# Autodesk Inventor assembly: Lens_mounted
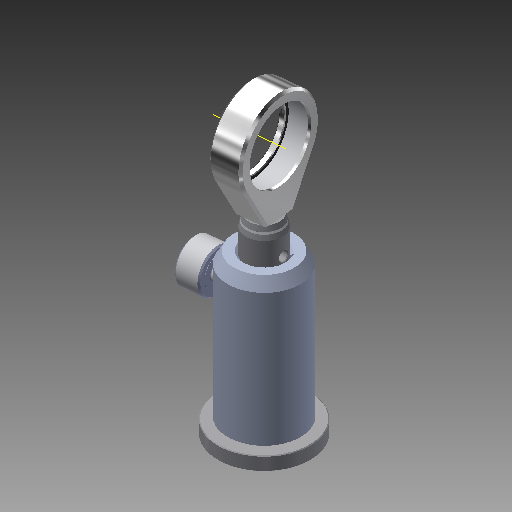
[picture p0: Inventor's stored thumbnail of the model, 512x512]
Saved by Autodesk Inventor 2017 SP1 (Build 210196100, 196)
## iProperties
Created: 2016-01-14
Part Number: Lens_mounted
Document SubType Name: Assembly
Designer: Conor Mow-Lowry
Author: Conor Mow-Lowry
## Documents named in this file (5)
- C:\Users\Sam\Documents\Inventor\outreach\portableMich\Lens_mounted.iam
- C:\Users\Sam\Documents\Inventor\outreach\portableMich\BE1_M-Step.ipt
- C:\Users\Sam\Documents\Inventor\outreach\portableMich\PH50V_M-Step.ipt
- C:\Users\Sam\Documents\Inventor\outreach\portableMich\TR50_M-Step.ipt
- C:\Users\Sam\Documents\Inventor\outreach\portableMich\LMR1_M-Step.ipt
## Components (4 placed, 4 different names)
1. BE1_M-Step:1 — Mate:1, Mate:2, Angle:1, Mate:7
2. PH50V_M-Step:1 — Mate:1, Mate:2, Mate:3, Angle:1, Angle:2
3. TR50_M-Step:1 — Mate:3, Mate:5, Mate:6, Angle:2, Angle:3
4. LMR1_M-Step:1 — Mate:5, Mate:6, Angle:3, Mate:7
## Relationships (9: Mate 6, Angle 3)
- Mate:1: BE1_M-Step:1 ↔ PH50V_M-Step:1
- Mate:2: BE1_M-Step:1 ↔ PH50V_M-Step:1
- Mate:3: PH50V_M-Step:1 ↔ TR50_M-Step:1
- Mate:5: TR50_M-Step:1 ↔ LMR1_M-Step:1
- Mate:6: TR50_M-Step:1 ↔ LMR1_M-Step:1
- Angle:1 (0 deg): BE1_M-Step:1 ↔ PH50V_M-Step:1
- Angle:2 (0 deg): PH50V_M-Step:1 ↔ TR50_M-Step:1
- Angle:3 (0 deg): TR50_M-Step:1 ↔ LMR1_M-Step:1
- Mate:7 (-88.1 mm): BE1_M-Step:1 ↔ LMR1_M-Step:1
